# Autodesk Inventor assembly: reference_magnet
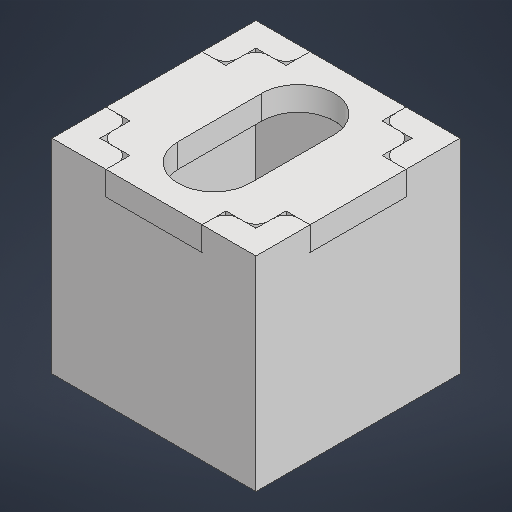
[picture p0: Inventor's stored thumbnail of the model, 512x512]
Saved by Autodesk Inventor 2026.1 (Build 301233020, 233B)
## iProperties
Created: 2025-11-29
Part Number: reference_magnet
Document SubType Name: Assembly
Designer: Carla Fernandez
Author: Carla Fernandez
## Documents named in this file (3)
- C:\Users\Carla Fernandez\Documents\GitHub\OSII_MINI_V2\CAD MODELS_screw_on\Calibration Tools\reference_magnet.iam
- C:\Users\Carla Fernandez\Documents\GitHub\OSII_MINI_V2\CAD MODELS_screw_on\Calibration Tools\reference_magnet_box.ipt
- C:\Users\Carla Fernandez\Documents\GitHub\OSII_MINI_V2\CAD MODELS_screw_on\Calibration Tools\reference_magnet_lid.ipt
## Components (2 placed, 2 different names)
1. reference_magnet_box:1 — Mate:1, Flush:1, Flush:2
2. reference_magnet_lid:1 — Mate:1, Flush:1, Flush:2
## Relationships (3: Flush 2, Mate 1)
- Mate:1: reference_magnet_box:1 ↔ reference_magnet_lid:1
- Flush:1: reference_magnet_box:1 ↔ reference_magnet_lid:1
- Flush:2: reference_magnet_box:1 ↔ reference_magnet_lid:1
